# Autodesk Inventor assembly: ASY GBK 1310 long wall shield 4
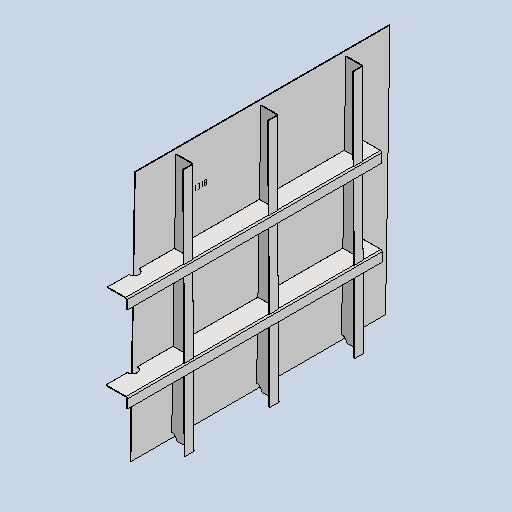
[picture p0: Inventor's stored thumbnail of the model, 512x512]
Saved by Autodesk Inventor 2026.2 (Build 302298010, 298A)
## iProperties
Created: 2026-05-07
Part Number: ASY GBK 1310 long wall shield 4
Document SubType Name: Assembly
Designer: pokla
Mass: 107756 g
Surface Area: 69611.7 cm^2
Volume: 13726.9 cm^3
Density: 7.85 g/cm^3
Stock Number: 1311
Author: admin
## Documents named in this file (6)
- C:\Users\admin\Desktop\GBK-Gubkinskiy\ASY GBK 1310 long wall shield 4.iam
- C:\Users\admin\Desktop\GBK-Gubkinskiy\07.1 GBK shield.ipt
- C:\Users\admin\Desktop\GBK-Gubkinskiy\GBK 0301 third rib.ipt
- C:\Users\admin\Desktop\GBK-Gubkinskiy\GBK 0302 stringer 7.ipt
- C:\Users\admin\Desktop\GBK-Gubkinskiy\GBK 0303 stringer 8.ipt
- C:\Users\admin\Desktop\GBK-Gubkinskiy\GBK 0101 main rib.ipt
## Components (6 placed, 4 different names)
1. GBK 0302 stringer 7.ipt:1
2. GBK 0303 stringer 8.ipt:1
3. 07.1 GBK shield.ipt:1
4. GBK 0301 third rib.ipt:1
5. GBK 0301 third rib.ipt:2
6. GBK 0301 third rib.ipt:3
## Component patterns: (3 elements, first: GBK 0301 third rib.ipt:1)
## Relationships (5: Mate 2, WeldJoint 2, Flush 1)
- [Flush] (254 mm): 07.1 GBK shield.ipt:1 ↔ GBK 0301 third rib.ipt:1
- [Mate]: 07.1 GBK shield.ipt:1 ↔ GBK 0301 third rib.ipt:1
- [Mate]: 07.1 GBK shield.ipt:1 ↔ GBK 0301 third rib.ipt:1
- [WeldJoint] (4 mm): GBK 0302 stringer 7.ipt:1 ↔ GBK 0301 third rib.ipt:1
- [WeldJoint] (4 mm): GBK 0303 stringer 8.ipt:1 ↔ GBK 0301 third rib.ipt:1
## Named parameters: Шаг_шпангоутов = 496.66667 mm
